# Autodesk Inventor assembly: dog clutch
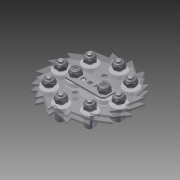
[picture p0: Inventor's stored thumbnail of the model, 180x180]
Saved by Autodesk Inventor 2014 SP1 (Build 180222100, 222)
## iProperties
Created: 2014-02-23
Part Number: dog clutch
Document SubType Name: Assembly
Designer: Ryan
Author: Ryan
## Documents named in this file (8)
- C:\Users\Ryan\Desktop\sw\toss up 4th robot\drive\ratchet dog clutch.iam
- C:\Users\Ryan\Desktop\sw\lib\Aperture VEX CAD Library\Hardware\8-32\8-32 nylock.ipt
- C:\Users\Ryan\Desktop\sw\toss up 4th robot\drive\ratchet test\HS 60 tooth dog clutch.ipt
- C:\Users\Ryan\Desktop\sw\lib\Aperture VEX CAD Library\Metal\Gussets\Lockbar.ipt
- C:\Users\Ryan\Desktop\sw\lib\Aperture VEX CAD Library\Spacers\thin\SPACER-0320-0250.ipt
- C:\Users\Ryan\Desktop\sw\lib\Aperture VEX CAD Library\Spacers\SPACER-0500-0125.ipt
- C:\Users\Ryan\Desktop\sw\lib\Aperture VEX CAD Library\Hardware\8-32\8-23_.750.ipt
- C:\Users\Ryan\Desktop\sw\lib\Aperture VEX CAD Library\Hardware\8-32\8-32_.500.ipt
## Components (42 placed, 7 different names)
1. HS 60 tooth dog clutch:1 — Mate:7, Mate:12, Flush:1, Flush:2, Mate:16, Mate:17, Mate:28, Mate:29, Mate:30
2. HS 60 tooth dog clutch:2 — Mate:15, Mate:16, Mate:17, Mate:25, Mate:26, Mate:27, Mate:43, Mate:46
3. Lockbar:1 — Mate:25, Mate:26, Mate:27, Mate:47, Mate:48, Mate:49, Mate:50
4. Lockbar:2 — Mate:28, Mate:29, Mate:30, Flush:3, Flush:4, Mate:44, Mate:45, Mate:52, Mate:53
5. SPACER-0500-0125:9 — Mate:43, Mate:44
6. SPACER-0500-0125:10 — Mate:45, Mate:46
7. 8-32_.500:1 — Mate:47, Mate:48, Mate:54
8. 8-32_.500:2 — Mate:49, Mate:50, Mate:51
9. 8-32 nylock:9 — Mate:51, Mate:52
10. 8-32 nylock:10 — Mate:53, Mate:54
11. 8-32 nylock:1 — Mate:12, Mate:22
12. 8-23_.750:1 — Mate:41, Mate:42
13. SPACER-0500-0125:1
14. SPACER-0320-0250:1 — Mate:7, Mate:15, Mate:22, Mate:41, Mate:42
15. 8-32 nylock:2
16. 8-23_.750:2
17. SPACER-0500-0125:2
18. SPACER-0320-0250:2
19. 8-32 nylock:3
20. 8-23_.750:3
21. SPACER-0500-0125:3
22. SPACER-0320-0250:3
23. 8-32 nylock:4
24. 8-23_.750:4
25. SPACER-0500-0125:4
26. SPACER-0320-0250:4
27. 8-32 nylock:5
28. 8-23_.750:5
29. SPACER-0500-0125:5
30. SPACER-0320-0250:5
31. 8-32 nylock:6
32. 8-23_.750:6
33. SPACER-0500-0125:6
34. SPACER-0320-0250:6
35. 8-32 nylock:7
36. 8-23_.750:7
37. SPACER-0500-0125:7
38. SPACER-0320-0250:7
39. 8-32 nylock:8
40. 8-23_.750:8
41. SPACER-0500-0125:8
42. SPACER-0320-0250:8
## Component patterns: (8 elements, first: 8-32 nylock:1 + 8-23_.750:1 + SPACER-0500-0125:1 + SPACER-0320-0250:1)
## Relationships (37: Mate 33, Flush 4)
- Mate:7: HS 60 tooth dog clutch:1 ↔ SPACER-0320-0250:1
- Mate:12: HS 60 tooth dog clutch:1 ↔ 8-32 nylock:1
- Flush:1 (1.5367 mm): HS 60 tooth dog clutch:1
- Flush:2 (1.5367 mm): HS 60 tooth dog clutch:1
- Mate:13
- Mate:14
- Mate:15: HS 60 tooth dog clutch:2 ↔ SPACER-0320-0250:1
- Mate:16: HS 60 tooth dog clutch:1 ↔ HS 60 tooth dog clutch:2
- Mate:17: HS 60 tooth dog clutch:1 ↔ HS 60 tooth dog clutch:2
- [Mate]: HS 60 tooth dog clutch:2 ↔ SPACER-0500-0125:1
- [Mate]: HS 60 tooth dog clutch:1 ↔ SPACER-0500-0125:1
- [Mate]: SPACER-0500-0125:1 ↔ SPACER-0320-0250:1
- Mate:22: 8-32 nylock:1 ↔ SPACER-0320-0250:1
- Mate:25: HS 60 tooth dog clutch:2 ↔ Lockbar:1
- Mate:26: HS 60 tooth dog clutch:2 ↔ Lockbar:1
- Mate:27: HS 60 tooth dog clutch:2 ↔ Lockbar:1
- Mate:28: HS 60 tooth dog clutch:1 ↔ Lockbar:2
- Mate:29: HS 60 tooth dog clutch:1 ↔ Lockbar:2
- Mate:30: HS 60 tooth dog clutch:1 ↔ Lockbar:2
- Flush:3 (1.6002 mm): Lockbar:2
- Flush:4 (1.6002 mm): Lockbar:2
- Mate:39
- Mate:40
- Mate:41: 8-23_.750:1 ↔ SPACER-0320-0250:1
- Mate:42: 8-23_.750:1 ↔ SPACER-0320-0250:1
- Mate:43: HS 60 tooth dog clutch:2 ↔ SPACER-0500-0125:9
- Mate:44: Lockbar:2 ↔ SPACER-0500-0125:9
- Mate:45: Lockbar:2 ↔ SPACER-0500-0125:10
- Mate:46: HS 60 tooth dog clutch:2 ↔ SPACER-0500-0125:10
- Mate:47: Lockbar:1 ↔ 8-32_.500:1
- Mate:48: Lockbar:1 ↔ 8-32_.500:1
- Mate:49: Lockbar:1 ↔ 8-32_.500:2
- Mate:50: Lockbar:1 ↔ 8-32_.500:2
- Mate:51: 8-32_.500:2 ↔ 8-32 nylock:9
- Mate:52: Lockbar:2 ↔ 8-32 nylock:9
- Mate:53: Lockbar:2 ↔ 8-32 nylock:10
- Mate:54: 8-32_.500:1 ↔ 8-32 nylock:10
